# Autodesk Inventor assembly: ax12
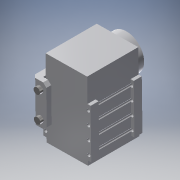
[picture p0: Inventor's stored thumbnail of the model, 180x180]
Saved by Autodesk Inventor 2017 SP1 (Build 210196100, 196)
## iProperties
Created: 2017-11-23
Part Number: ax12
Document SubType Name: Assembly
Designer: Biscuit
Author: Biscuit
## Documents named in this file (8)
- C:\Users\Cortman\Google Drive\ENSEIRB\EIRBOT\COUPE 2018\Cubes\ax12.iam
- C:\Users\Cortman\Google Drive\ENSEIRB\EIRBOT\COUPE 2018\Cubes\ax12.ipt
- C:\Users\Cortman\Google Drive\ENSEIRB\EIRBOT\COUPE 2018\Cubes\axe_ax12.ipt
- C:\Users\Cortman\Google Drive\ENSEIRB\EIRBOT\COUPE 2018\Cubes\fixation_ax12.ipt
- C:\Users\Cortman\Google Drive\ENSEIRB\EIRBOT\COUPE 2018\Cubes\ax12\Design Accelerator\Arbre1.iam
- C:\Users\Cortman\Google Drive\ENSEIRB\EIRBOT\COUPE 2018\Cubes\ax12\Design Accelerator\Arbre2.iam
- C:\Users\Cortman\Google Drive\ENSEIRB\EIRBOT\COUPE 2018\Cubes\ax12\Design Accelerator\Arbre3.iam
- C:\Users\Cortman\Google Drive\ENSEIRB\EIRBOT\COUPE 2018\Cubes\ax12\Design Accelerator\Arbre4.iam
## Components (7 placed, 4 different names)
1. ax12:1 — Mate:1, Mate:2, Placage:3, Placage:4, Placage:5
2. axe_ax12:1 — Mate:1, Mate:2
3. fixation_ax12:2 — Placage:3, Placage:4, Placage:5, Placage:6, Placage:7, Angle:1, Placage:8, Placage:9, Angle:2, Placage:10, Placage:11, Angle:3, Placage:12, Placage:13, Angle:4
4. Arbre:1 [sub-assembly] — Placage:6, Placage:7, Angle:1
5. Arbre:2 [sub-assembly] — Placage:8, Placage:9, Angle:2
6. Arbre:3 [sub-assembly] — Placage:10, Placage:11, Angle:3
7. Arbre:4 [sub-assembly] — Placage:12, Placage:13, Angle:4
## Relationships (17: Mate 13, Angle 4)
- Mate:1: ax12:1 ↔ axe_ax12:1
- Mate:2 (0.5 mm): ax12:1 ↔ axe_ax12:1
- Placage:3 [Mate]: ax12:1 ↔ fixation_ax12:2
- Placage:4 [Mate]: ax12:1 ↔ fixation_ax12:2
- Placage:5 [Mate]: ax12:1 ↔ fixation_ax12:2
- Placage:6 [Mate]: fixation_ax12:2 ↔ Arbre:1
- Placage:7 [Mate] (2 mm): fixation_ax12:2 ↔ Arbre:1
- Angle:1 (0 deg): fixation_ax12:2 ↔ Arbre:1
- Placage:8 [Mate]: fixation_ax12:2 ↔ Arbre:2
- Placage:9 [Mate] (2 mm): fixation_ax12:2 ↔ Arbre:2
- Angle:2 (0 deg): fixation_ax12:2 ↔ Arbre:2
- Placage:10 [Mate]: fixation_ax12:2 ↔ Arbre:3
- Placage:11 [Mate] (2 mm): fixation_ax12:2 ↔ Arbre:3
- Angle:3 (0 deg): fixation_ax12:2 ↔ Arbre:3
- Placage:12 [Mate]: fixation_ax12:2 ↔ Arbre:4
- Placage:13 [Mate] (2 mm): fixation_ax12:2 ↔ Arbre:4
- Angle:4 (0 deg): fixation_ax12:2 ↔ Arbre:4
